# Autodesk Inventor assembly: Pipe Support - Unistrut PS06-01
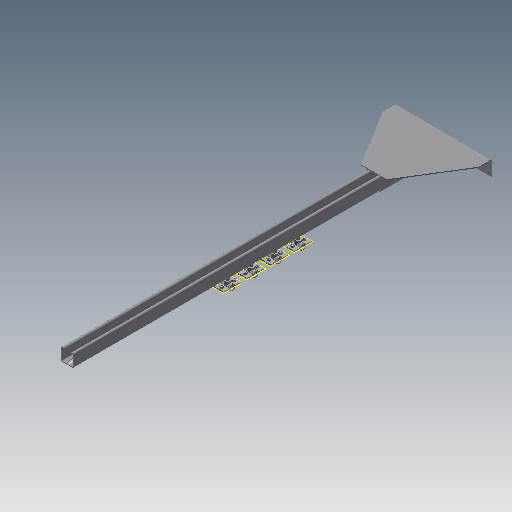
[picture p0: Inventor's stored thumbnail of the model, 512x512]
Saved by Autodesk Inventor 2020 (Build 240152000, 152)
## iProperties
Created: 2009-08-10
Part Number: Pipe Support - Unistrut PS06-01
Document SubType Name: Assembly
Designer: Demir Ali
Description: Pipe Support
Stock Number: NA
Author: Demir Ali
Title: Purchased Part
Revision Number: A
## Documents named in this file (4)
- C:\Users\hallc\Desktop\Process Equipment\Workspace\Options\Pipe Support - Unistrut PS06-01.iam
- C:\Users\hallc\Desktop\Process Equipment\Workspace\Supplier Content\P2348-S1-Unistrut.ipt
- C:\Users\hallc\Desktop\Process Equipment\Workspace\Supplier Content\P1000 x 1000.ipt
- C:\Users\hallc\Desktop\Process Equipment\Workspace\Supplier Content\Pipe Clamp - 25.ipt
## Components (6 placed, 3 different names)
1. P2348-S1-Unistrut:1 — Mate:2, Mate:3, Mate:4
2. P1000 x 1000:1 — Mate:2, Mate:3, Mate:4, Rigid:1
3. Pipe Clamp - 25:1 — Rigid:1
4. Pipe Clamp - 25:2
5. Pipe Clamp - 25:3
6. Pipe Clamp - 25:4
## Component patterns: (4 elements, first: Pipe Clamp - 25:1)
## Relationships (4: Mate 3, WeldJoint 1)
- Mate:2: P2348-S1-Unistrut:1 ↔ P1000 x 1000:1
- Mate:3: P2348-S1-Unistrut:1 ↔ P1000 x 1000:1
- Mate:4: P2348-S1-Unistrut:1 ↔ P1000 x 1000:1
- Rigid:1 [WeldJoint]: P1000 x 1000:1 ↔ Pipe Clamp - 25:1
